# Autodesk Inventor assembly: LegConstruction
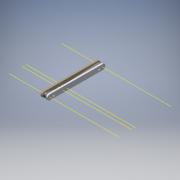
[picture p0: Inventor's stored thumbnail of the model, 180x180]
Saved by Autodesk Inventor 2019.1 (Build 231200000, 200)
## iProperties
Created: 2018-10-30
Part Number: LegConstruction
Material: Generisch
Document SubType Name: Assembly
Designer: JochenAlt
Author: JochenAlt
## Documents named in this file (3)
- D:\Projects\Ondine\CAD\Leg\LegConstruction.iam
- D:\Projects\Ondine\CAD\Leg\LegConstruction\Konstruktions-Assistent\Übertragung des Zahnriemens1.iam
- D:\Projects\Ondine\CAD\Leg\Thigh.ipt
## Components (2 placed, 2 different names)
1. Thigh:1 — Passend:1, Passend:2, Passend:3, Passend:4
2. Übertragung des Zahnriemens:1 [sub-assembly] — Passend:4
## Relationships (4: Mate 4)
- Passend:1 [Mate]: Thigh:1
- Passend:2 [Mate]: Thigh:1
- Passend:3 [Mate]: Thigh:1
- Passend:4 [Mate] (0.5 mm): Thigh:1 ↔ Übertragung des Zahnriemens:1
